# Autodesk Inventor assembly: Система подачи и забора проволоки
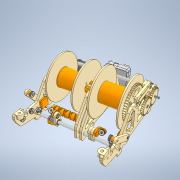
[picture p0: Inventor's stored thumbnail of the model, 180x180]
Saved by Autodesk Inventor 2021.1 (Build 251245010, 245A)
## iProperties
Created: 2026-04-13
Part Number: Система подачи и забора проволоки
Document SubType Name: Assembly
Designer: Андрей Тарасов
Author: Андрей Тарасов
## Documents named in this file (49)
- G:\04. Inventor\024. EDM 3.0\Система подачи и забора  проволоки\Система подачи и забора проволоки.iam
- G:\04. Inventor\024. EDM 3.0\Система подачи и забора  проволоки\Барабан катушки.ipt
- G:\04. Inventor\024. EDM 3.0\Система подачи и забора  проволоки\Бортик катушки.ipt
- G:\04. Inventor\024. EDM 3.0\Система подачи и забора  проволоки\Бортик внутренний.ipt
- G:\04. Inventor\024. EDM 3.0\Система подачи и забора  проволоки\Конусный барабан катушки.ipt
- G:\04. Inventor\024. EDM 3.0\Система подачи и забора  проволоки\Бортик конусной катушки.ipt
- G:\04. Inventor\024. EDM 3.0\Система подачи и забора  проволоки\Бортик внутренний (конусной катушки).ipt
- G:\04. Inventor\024. EDM 3.0\Система подачи и забора  проволоки\Вал катушки.ipt
- G:\04. Inventor\024. EDM 3.0\Система подачи и забора  проволоки\Опора катушки.ipt
- G:\04. Inventor\024. EDM 3.0\Система подачи и забора  проволоки\Опора катушки (врунтренняя).ipt
- G:\04. Inventor\024. EDM 3.0\Система подачи и забора  проволоки\Подшипник (8х12х3.5).ipt
- G:\04. Inventor\024. EDM 3.0\Система подачи и забора  проволоки\Вал шестерни.ipt
- G:\04. Inventor\024. EDM 3.0\Система подачи и забора  проволоки\Шестерня катушки.ipt
- G:\04. Inventor\024. EDM 3.0\Система подачи и забора  проволоки\Промежуточная шестерня (малая).ipt
- G:\04. Inventor\024. EDM 3.0\Система подачи и забора  проволоки\Рычаг фиксатора 1.ipt
- G:\04. Inventor\024. EDM 3.0\Система подачи и забора  проволоки\U-подшипник.ipt
- G:\04. Inventor\024. EDM 3.0\Система подачи и забора  проволоки\Рычаг натяжителя.ipt
- G:\04. Inventor\024. EDM 3.0\Система подачи и забора  проволоки\Петля ролика.ipt
- G:\04. Inventor\024. EDM 3.0\Система подачи и забора  проволоки\Крепление петли.ipt
- G:\04. Inventor\024. EDM 3.0\Система подачи и забора  проволоки\Крепление шкива.ipt
- G:\04. Inventor\024. EDM 3.0\Система подачи и забора  проволоки\Фиксатор трубки.ipt
- G:\04. Inventor\024. EDM 3.0\Система подачи и забора  проволоки\Трубка опоры (8 мм).ipt
- G:\04. Inventor\024. EDM 3.0\Система подачи и забора  проволоки\Петля ролика_MIR.ipt
- G:\04. Inventor\024. EDM 3.0\Система подачи и забора  проволоки\Линейный подшипник.ipt
- G:\04. Inventor\024. EDM 3.0\Система подачи и забора  проволоки\Крепление линейного подшипника.ipt
- G:\04. Inventor\024. EDM 3.0\Система подачи и забора  проволоки\Проставка катушки левая.ipt
- G:\04. Inventor\024. EDM 3.0\Система подачи и забора  проволоки\Проставка катушки правая.ipt
- G:\04. Inventor\024. EDM 3.0\Система подачи и забора  проволоки\Фиксатор левый.iam
- G:\04. Inventor\024. EDM 3.0\Система подачи и забора  проволоки\Фиксатор правый.iam
- G:\04. Inventor\024. EDM 3.0\Система подачи и забора  проволоки\Проставка шестерни.ipt
- G:\04. Inventor\024. EDM 3.0\Система подачи и забора  проволоки\Вал катушки (левой).ipt
- G:\04. Inventor\024. EDM 3.0\Система подачи и забора  проволоки\Вал шестерни (левой).ipt
- G:\04. Inventor\024. EDM 3.0\Система подачи и забора  проволоки\Проставка рычага натяжителя.ipt
- G:\04. Inventor\024. EDM 3.0\Система подачи и забора  проволоки\Бесконечный винт.ipt
- G:\04. Inventor\024. EDM 3.0\Система подачи и забора  проволоки\Бегунок.ipt
- G:\04. Inventor\024. EDM 3.0\Система подачи и забора  проволоки\Кольцо линейного подшипника.ipt
- G:\04. Inventor\024. EDM 3.0\Система подачи и забора  проволоки\Трубка винта.ipt
- G:\04. Inventor\024. EDM 3.0\Система подачи и забора  проволоки\AS5600.ipt
- G:\04. Inventor\024. EDM 3.0\Система подачи и забора  проволоки\Nema-17.ipt
- G:\04. Inventor\024. EDM 3.0\Система подачи и забора  проволоки\Шестерня мотора.ipt
- G:\04. Inventor\024. EDM 3.0\Система подачи и забора  проволоки\Шестерня промежуточная (большая).ipt
- G:\04. Inventor\024. EDM 3.0\Система подачи и забора  проволоки\Stepper 28BYJ-48.ipt
- G:\04. Inventor\024. EDM 3.0\Система подачи и забора  проволоки\Трубка рычага.ipt
- G:\04. Inventor\024. EDM 3.0\Система подачи и забора  проволоки\Шпунтик.ipt
- G:\04. Inventor\024. EDM 3.0\Система подачи и забора  проволоки\Шайба датчика.ipt
- G:\04. Inventor\024. EDM 3.0\Система подачи и забора  проволоки\Плата.ipt
- G:\04. Inventor\024. EDM 3.0\Система подачи и забора  проволоки\Корпус платы.ipt
- G:\04. Inventor\024. EDM 3.0\Система подачи и забора  проволоки\Крышка корпуса платы.ipt
- G:\04. Inventor\024. EDM 3.0\Колпачок датчика.ipt
## Components (93 placed, 48 different names)
1. Барабан катушки:1 — Совмещение:1, Совмещение:2, Заподлицо:1, Заподлицо:2, Совмещение:8, Совмещение:9
2. Бортик катушки:1 — Совмещение:1, Заподлицо:1, Заподлицо:6, Заподлицо:12, Совмещение:20, Совмещение:53, Совмещение:54
3. Бортик катушки:2 — Совмещение:2, Заподлицо:2, Заподлицо:7, Совмещение:63
4. Бортик катушки:3 — Совмещение:10, Заподлицо:8, Заподлицо:9, Совмещение:28, Совмещение:124, Заподлицо:50
5. Бортик внутренний:1 — Совмещение:12, Заподлицо:9, Совмещение:165
6. Бортик внутренний:2 — Совмещение:9, Заподлицо:7
7. Бортик внутренний:3 — Совмещение:8, Заподлицо:6, Совмещение:18
8. Конусный барабан катушки:1 — Совмещение:10, Заподлицо:8, Совмещение:12, Совмещение:15, Заподлицо:10, Совмещение:17
9. Бортик конусной катушки:1 — Совмещение:16, Совмещение:17, Совмещение:64
10. Бортик внутренний (конусной катушки):1 — Совмещение:15, Заподлицо:10, Совмещение:16
11. Вал катушки:1 — Совмещение:18, Заподлицо:12, Совмещение:22, Совмещение:52
12. Опора катушки:1 — Совмещение:20, Совмещение:22, Совмещение:46, Совмещение:47, Заподлицо:15, Заподлицо:16, Совмещение:73, Заподлицо:30, Совмещение:93, Совмещение:94, Совмещение:96, Совмещение:97, Совмещение:98, Совмещение:99, Совмещение:100, Заподлицо:31, Заподлицо:32, Совмещение:102, Совмещение:103, Совмещение:107, Заподлицо:33, Совмещение:111, Совмещение:145, Совмещение:164, Совмещение:206, Совмещение:207, Совмещение:212, Совмещение:216, Совмещение:217, Совмещение:220, Совмещение:221, Совмещение:238, Совмещение:244, Совмещение:247, Совмещение:248, Совмещение:259
13. Опора катушки:2 — Совмещение:28, Совмещение:44, Совмещение:45, Заподлицо:17, Заподлицо:18, Заподлицо:34, Заподлицо:37, Совмещение:119, Совмещение:120, Совмещение:140, Совмещение:141, Совмещение:142, Совмещение:146, Совмещение:154, Совмещение:155, Заподлицо:40, Совмещение:166, Совмещение:167, Совмещение:168, Совмещение:169, Совмещение:170, Совмещение:171, Совмещение:172, Совмещение:175, Заподлицо:42, Совмещение:176, Совмещение:177, Совмещение:190, Совмещение:195, Совмещение:196, Заподлицо:47, Заподлицо:49, Совмещение:204, Совмещение:209, Совмещение:210, Совмещение:213, Совмещение:218, Совмещение:219, Совмещение:222, Совмещение:223, Совмещение:229, Совмещение:231, Заподлицо:53, Совмещение:239, Совмещение:240, Совмещение:241, Заподлицо:58, Заподлицо:59, Совмещение:249, Совмещение:250, Совмещение:251, Совмещение:252, Совмещение:260
14. Подшипник (8х12х3.5):1 — Совмещение:46, Заподлицо:16
15. Подшипник (8х12х3.5):2 — Совмещение:47, Заподлицо:15, Совмещение:50
16. Подшипник (8х12х3.5):3 — Совмещение:44, Заподлицо:18
17. Подшипник (8х12х3.5):4 — Совмещение:45, Заподлицо:17, Совмещение:228
18. Вал шестерни:1 — Совмещение:50, Совмещение:51, Совмещение:54, Совмещение:227
19. Шестерня катушки:1 — Совмещение:52, Совмещение:53
20. Промежуточная шестерня (малая):1 — Совмещение:51, Совмещение:164
21. Опора катушки (врунтренняя):1 — Совмещение:64, Совмещение:109, Совмещение:139, Совмещение:143, Совмещение:144, Совмещение:150, Совмещение:197, Заподлицо:48, Совмещение:242, Совмещение:243, Совмещение:258, Заподлицо:60
22. Опора катушки (врунтренняя):2 — Совмещение:63, Совмещение:108, Совмещение:114, Совмещение:242
23. U-подшипник:1 — Совмещение:74, Совмещение:75
24. U-подшипник:2 — Совмещение:98, Совмещение:99
25. U-подшипник:3 — Совмещение:91, Совмещение:92
26. Подшипник (8х12х3.5):5 — Совмещение:100, Заподлицо:31, Совмещение:101
27. Рычаг натяжителя:1 — Совмещение:73, Совмещение:74, Совмещение:75, Совмещение:101, Совмещение:183, Совмещение:184, Совмещение:236, Заподлицо:56, Заподлицо:57
28. Петля ролика:1 — Совмещение:104, Совмещение:105, Совмещение:106, Совмещение:113
29. Крепление петли:1 — Совмещение:104, Совмещение:110, Совмещение:111, Совмещение:113, Совмещение:114, Совмещение:115, Заподлицо:35, Совмещение:117
30. U-подшипник:4 — Совмещение:105, Совмещение:106
31. Подшипник (8х12х3.5):6 — Совмещение:115, Заподлицо:35
32. Подшипник (8х12х3.5):7 — Совмещение:118, Заподлицо:36
33. Крепление шкива:1 — Совмещение:91, Совмещение:92, Заподлицо:30, Совмещение:93, Совмещение:94
34. U-подшипник:5 — Совмещение:96, Совмещение:97
35. Фиксатор трубки:1 — Заподлицо:32, Совмещение:102, Совмещение:103
36. Трубка опоры (8 мм):1 — Совмещение:107, Заподлицо:33, Совмещение:108, Совмещение:109, Заподлицо:34, Совмещение:110, Совмещение:116, Совмещение:131, Совмещение:204
37. Крепление петли:2 — Совмещение:116, Совмещение:117, Совмещение:118, Заподлицо:36
38. Крепление шкива:2 — Заподлицо:37, Совмещение:119, Совмещение:120, Совмещение:121, Совмещение:122
39. U-подшипник:6 — Совмещение:121, Совмещение:122
40. Шестерня катушки:2 — Совмещение:124, Совмещение:232
41. Петля ролика_MIR:1 — Совмещение:129, Совмещение:130, Совмещение:137, Совмещение:138
42. U-подшипник:7 — Совмещение:129, Совмещение:130
43. Линейный подшипник:1 — Совмещение:131, Совмещение:133, Совмещение:192, Заподлицо:44, Заподлицо:45
44. Крепление линейного подшипника:2 — Совмещение:133, Совмещение:137, Совмещение:138, Заподлицо:45, Совмещение:195, Совмещение:198, Заподлицо:46
45. Проставка катушки левая:1 — Совмещение:140, Совмещение:141, Совмещение:142
46. Проставка катушки правая:1 — Совмещение:139, Совмещение:143, Совмещение:144
47. Фиксатор левый:1 [sub-assembly] — Совмещение:145
48. Фиксатор правый:1 [sub-assembly] — Совмещение:146, Совмещение:156
49. Фиксатор левый:2 [sub-assembly] — Совмещение:150, Совмещение:151, Совмещение:152, Совмещение:153, Совмещение:253
50. Рычаг фиксатора 1:1 — Совмещение:151, Совмещение:152, Совмещение:153
51. Проставка шестерни:1 — Совмещение:154, Совмещение:155, Совмещение:156, Совмещение:160
52. Промежуточная шестерня (малая):2 — Совмещение:160
53. Вал катушки (левой):1 — Совмещение:165, Заподлицо:40, Совмещение:166, Совмещение:232
54. U-подшипник:8 — Совмещение:167, Совмещение:169
55. U-подшипник:9 — Совмещение:168, Совмещение:170
56. Рычаг натяжителя:2 — Совмещение:171, Совмещение:172, Совмещение:173, Совмещение:174, Совмещение:181, Совмещение:182, Совмещение:234, Заподлицо:54, Заподлицо:55
57. U-подшипник:10 — Совмещение:173, Совмещение:174
58. Подшипник (8х12х3.5):8 — Совмещение:175, Заподлицо:53
59. Фиксатор трубки:2 — Заподлицо:42, Совмещение:176, Совмещение:177
60. Вал шестерни (левой):1 — Совмещение:224, Совмещение:228, Заподлицо:52
61. Проставка рычага натяжителя:1 — Совмещение:181, Совмещение:182
62. Проставка рычага натяжителя:2 — Совмещение:183, Совмещение:184
63. Бесконечный винт:1 — Совмещение:190, Совмещение:193, Заподлицо:50
64. Бегунок:1 — Совмещение:193, Совмещение:194
65. Кольцо линейного подшипника:1 — Совмещение:192, Заподлицо:44, Совмещение:194
66. Подшипник (8х12х3.5):9 — Совмещение:196, Заподлицо:47, Совмещение:199
67. Подшипник (8х12х3.5):10 — Совмещение:198, Заподлицо:46
68. Подшипник (8х12х3.5):11 — Совмещение:197, Заподлицо:48
69. Трубка винта:1 — Совмещение:199, Заподлицо:49, Совмещение:230
70. AS5600:1 — Совмещение:206, Совмещение:207, Совмещение:238, Совмещение:245, Совмещение:246, Совмещение:263, Совмещение:264
71. AS5600:2 — Совмещение:209, Совмещение:210, Совмещение:239, Совмещение:261, Совмещение:262
72. Nema-17:1 — Совмещение:213, Совмещение:218, Совмещение:219, Совмещение:225
73. Nema-17:2 — Совмещение:212, Совмещение:216, Совмещение:217, Совмещение:226
74. Шестерня мотора:1 — Совмещение:221, Совмещение:226
75. Шестерня мотора:2 — Совмещение:222, Совмещение:225
76. Шестерня промежуточная (большая):1 — Совмещение:220, Совмещение:227
77. Шестерня промежуточная (большая):2 — Совмещение:223, Совмещение:224, Заподлицо:52
78. Stepper 28BYJ-48:1 — Совмещение:229, Совмещение:230, Совмещение:231
79. Трубка рычага:1 — Совмещение:236, Заподлицо:56, Совмещение:237
80. Шпунтик:1 — Заподлицо:55, Совмещение:235
81. Трубка рычага:2 — Совмещение:234, Заподлицо:54, Совмещение:235
82. Шпунтик:2 — Заподлицо:57, Совмещение:237
83. Трубка опоры (8 мм):2 — Совмещение:241, Заподлицо:59, Совмещение:243, Совмещение:244
84. Трубка опоры (8 мм):3 — Совмещение:240, Заподлицо:58, Совмещение:253
85. Шайба датчика:1 — Совмещение:250, Совмещение:252
86. Шайба датчика:2 — Совмещение:249, Совмещение:251
87. Шайба датчика:3 — Совмещение:245, Совмещение:247
88. Шайба датчика:4 — Совмещение:246, Совмещение:248
89. Плата:1 — Совмещение:254
90. Корпус платы:1 — Совмещение:254, Совмещение:255, Совмещение:256, Совмещение:257, Совмещение:258, Заподлицо:60
91. Крышка корпуса платы:1 — Совмещение:255, Совмещение:256, Совмещение:257
92. Колпачок датчика:1 — Совмещение:260, Совмещение:261, Совмещение:262
93. Колпачок датчика:2 — Совмещение:259, Совмещение:263, Совмещение:264
## Relationships (200: Mate 162, Flush 38)
- Совмещение:1 [Mate]: Барабан катушки:1 ↔ Бортик катушки:1
- Совмещение:2 [Mate]: Барабан катушки:1 ↔ Бортик катушки:2
- Заподлицо:1 [Flush]: Барабан катушки:1 ↔ Бортик катушки:1
- Заподлицо:2 [Flush]: Барабан катушки:1 ↔ Бортик катушки:2
- Совмещение:8 [Mate]: Барабан катушки:1 ↔ Бортик внутренний:3
- Совмещение:9 [Mate]: Барабан катушки:1 ↔ Бортик внутренний:2
- Заподлицо:6 [Flush]: Бортик катушки:1 ↔ Бортик внутренний:3
- Заподлицо:7 [Flush]: Бортик катушки:2 ↔ Бортик внутренний:2
- Совмещение:10 [Mate]: Бортик катушки:3 ↔ Конусный барабан катушки:1
- Заподлицо:8 [Flush]: Бортик катушки:3 ↔ Конусный барабан катушки:1
- Совмещение:12 [Mate]: Бортик внутренний:1 ↔ Конусный барабан катушки:1
- Заподлицо:9 [Flush]: Бортик катушки:3 ↔ Бортик внутренний:1
- Совмещение:15 [Mate]: Конусный барабан катушки:1 ↔ Бортик внутренний (конусной катушки):1
- Заподлицо:10 [Flush] (4 mm): Конусный барабан катушки:1 ↔ Бортик внутренний (конусной катушки):1
- Совмещение:16 [Mate]: Бортик конусной катушки:1 ↔ Бортик внутренний (конусной катушки):1
- Совмещение:17 [Mate]: Конусный барабан катушки:1 ↔ Бортик конусной катушки:1
- Совмещение:18 [Mate]: Бортик внутренний:3 ↔ Вал катушки:1
- Заподлицо:12 [Flush] (-13 mm): Бортик катушки:1 ↔ Вал катушки:1
- Совмещение:20 [Mate] (7 mm): Бортик катушки:1 ↔ Опора катушки:1
- Совмещение:22 [Mate]: Вал катушки:1 ↔ Опора катушки:1
- Совмещение:28 [Mate] (20 mm): Бортик катушки:3 ↔ Опора катушки:2
- Совмещение:44 [Mate]: Опора катушки:2 ↔ Подшипник (8х12х3.5):3
- Совмещение:45 [Mate]: Опора катушки:2 ↔ Подшипник (8х12х3.5):4
- Совмещение:46 [Mate]: Опора катушки:1 ↔ Подшипник (8х12х3.5):1
- Совмещение:47 [Mate]: Опора катушки:1 ↔ Подшипник (8х12х3.5):2
- Заподлицо:15 [Flush] (-0.5 mm): Опора катушки:1 ↔ Подшипник (8х12х3.5):2
- Заподлицо:16 [Flush] (-0.5 mm): Опора катушки:1 ↔ Подшипник (8х12х3.5):1
- Заподлицо:17 [Flush] (-0.5 mm): Опора катушки:2 ↔ Подшипник (8х12х3.5):4
- Заподлицо:18 [Flush] (-0.5 mm): Опора катушки:2 ↔ Подшипник (8х12х3.5):3
- Совмещение:50 [Mate]: Подшипник (8х12х3.5):2 ↔ Вал шестерни:1
- Совмещение:51 [Mate]: Вал шестерни:1 ↔ Промежуточная шестерня (малая):1
- Совмещение:52 [Mate]: Вал катушки:1 ↔ Шестерня катушки:1
- Совмещение:53 [Mate]: Бортик катушки:1 ↔ Шестерня катушки:1
- Совмещение:54 [Mate] (0.5 mm): Бортик катушки:1 ↔ Вал шестерни:1
- Совмещение:63 [Mate] (1 mm): Бортик катушки:2 ↔ Опора катушки (врунтренняя):2
- Совмещение:64 [Mate] (15 mm): Бортик конусной катушки:1 ↔ Опора катушки (врунтренняя):1
- Совмещение:73 [Mate] (0.5 mm): Опора катушки:1 ↔ Рычаг натяжителя:1
- Совмещение:74 [Mate]: U-подшипник:1 ↔ Рычаг натяжителя:1
- Совмещение:75 [Mate] (7 mm): U-подшипник:1 ↔ Рычаг натяжителя:1
- Совмещение:91 [Mate]: U-подшипник:3 ↔ Крепление шкива:1
- Совмещение:92 [Mate] (0.5 mm): U-подшипник:3 ↔ Крепление шкива:1
- Заподлицо:30 [Flush]: Опора катушки:1 ↔ Крепление шкива:1
- Совмещение:93 [Mate]: Опора катушки:1 ↔ Крепление шкива:1
- Совмещение:94 [Mate]: Опора катушки:1 ↔ Крепление шкива:1
- Совмещение:96 [Mate]: Опора катушки:1 ↔ U-подшипник:5
- Совмещение:97 [Mate] (0.5 mm): Опора катушки:1 ↔ U-подшипник:5
- Совмещение:98 [Mate]: Опора катушки:1 ↔ U-подшипник:2
- Совмещение:99 [Mate] (0.5 mm): Опора катушки:1 ↔ U-подшипник:2
- Совмещение:100 [Mate]: Опора катушки:1 ↔ Подшипник (8х12х3.5):5
- Заподлицо:31 [Flush]: Опора катушки:1 ↔ Подшипник (8х12х3.5):5
- Совмещение:101 [Mate]: Подшипник (8х12х3.5):5 ↔ Рычаг натяжителя:1
- Заподлицо:32 [Flush]: Опора катушки:1 ↔ Фиксатор трубки:1
- Совмещение:102 [Mate]: Опора катушки:1 ↔ Фиксатор трубки:1
- Совмещение:103 [Mate]: Опора катушки:1 ↔ Фиксатор трубки:1
- Совмещение:104 [Mate]: Петля ролика:1 ↔ Крепление петли:1
- Совмещение:105 [Mate]: Петля ролика:1 ↔ U-подшипник:4
- Совмещение:106 [Mate]: Петля ролика:1 ↔ U-подшипник:4
- Совмещение:107 [Mate]: Опора катушки:1 ↔ Трубка опоры (8 мм):1
- Заподлицо:33 [Flush]: Опора катушки:1 ↔ Трубка опоры (8 мм):1
- Совмещение:108 [Mate]: Опора катушки (врунтренняя):2 ↔ Трубка опоры (8 мм):1
- Совмещение:109 [Mate]: Опора катушки (врунтренняя):1 ↔ Трубка опоры (8 мм):1
- Заподлицо:34 [Flush]: Опора катушки:2 ↔ Трубка опоры (8 мм):1
- Совмещение:110 [Mate]: Крепление петли:1 ↔ Трубка опоры (8 мм):1
- Совмещение:111 [Mate]: Опора катушки:1 ↔ Крепление петли:1
- Совмещение:113 [Mate] (0.5 mm): Петля ролика:1 ↔ Крепление петли:1
- Совмещение:114 [Mate] (21 mm): Опора катушки (врунтренняя):2 ↔ Крепление петли:1
- Совмещение:115 [Mate]: Крепление петли:1 ↔ Подшипник (8х12х3.5):6
- Заподлицо:35 [Flush]: Крепление петли:1 ↔ Подшипник (8х12х3.5):6
- Совмещение:116 [Mate]: Трубка опоры (8 мм):1 ↔ Крепление петли:2
- Совмещение:117 [Mate]: Крепление петли:1 ↔ Крепление петли:2
- Совмещение:118 [Mate]: Подшипник (8х12х3.5):7 ↔ Крепление петли:2
- Заподлицо:36 [Flush]: Подшипник (8х12х3.5):7 ↔ Крепление петли:2
- Заподлицо:37 [Flush]: Опора катушки:2 ↔ Крепление шкива:2
- Совмещение:119 [Mate]: Опора катушки:2 ↔ Крепление шкива:2
- Совмещение:120 [Mate]: Опора катушки:2 ↔ Крепление шкива:2
- Совмещение:121 [Mate]: Крепление шкива:2 ↔ U-подшипник:6
- Совмещение:122 [Mate] (0.5 mm): Крепление шкива:2 ↔ U-подшипник:6
- Совмещение:124 [Mate]: Бортик катушки:3 ↔ Шестерня катушки:2
- Совмещение:129 [Mate]: Петля ролика_MIR:1 ↔ U-подшипник:7
- Совмещение:130 [Mate]: Петля ролика_MIR:1 ↔ U-подшипник:7
- Совмещение:131 [Mate]: Трубка опоры (8 мм):1 ↔ Линейный подшипник:1
- Совмещение:133 [Mate]: Линейный подшипник:1 ↔ Крепление линейного подшипника:2
- Совмещение:137 [Mate]: Петля ролика_MIR:1 ↔ Крепление линейного подшипника:2
- Совмещение:138 [Mate] (0.5 mm): Петля ролика_MIR:1 ↔ Крепление линейного подшипника:2
- Совмещение:139 [Mate]: Опора катушки (врунтренняя):1 ↔ Проставка катушки правая:1
- Совмещение:140 [Mate]: Опора катушки:2 ↔ Проставка катушки левая:1
- Совмещение:141 [Mate]: Опора катушки:2 ↔ Проставка катушки левая:1
- Совмещение:142 [Mate]: Опора катушки:2 ↔ Проставка катушки левая:1
- Совмещение:143 [Mate]: Опора катушки (врунтренняя):1 ↔ Проставка катушки правая:1
- Совмещение:144 [Mate]: Опора катушки (врунтренняя):1 ↔ Проставка катушки правая:1
- Совмещение:145 [Mate]: Опора катушки:1 ↔ Фиксатор левый:1
- Совмещение:146 [Mate]: Опора катушки:2 ↔ Фиксатор правый:1
- Совмещение:150 [Mate] (0.5 mm): Опора катушки (врунтренняя):1 ↔ Фиксатор левый:2
- Совмещение:151 [Mate]: Фиксатор левый:2 ↔ Рычаг фиксатора 1:1
- Совмещение:152 [Mate]: Фиксатор левый:2 ↔ Рычаг фиксатора 1:1
- Совмещение:153 [Mate]: Фиксатор левый:2 ↔ Рычаг фиксатора 1:1
- Совмещение:154 [Mate]: Опора катушки:2 ↔ Проставка шестерни:1
- Совмещение:155 [Mate]: Опора катушки:2 ↔ Проставка шестерни:1
- Совмещение:156 [Mate]: Фиксатор правый:1 ↔ Проставка шестерни:1
- Совмещение:160 [Mate] (0.5 mm): Проставка шестерни:1 ↔ Промежуточная шестерня (малая):2
- Совмещение:164 [Mate] (0.5 mm): Опора катушки:1 ↔ Промежуточная шестерня (малая):1
- Совмещение:165 [Mate]: Бортик внутренний:1 ↔ Вал катушки (левой):1
- Заподлицо:40 [Flush]: Опора катушки:2 ↔ Вал катушки (левой):1
- Совмещение:166 [Mate]: Опора катушки:2 ↔ Вал катушки (левой):1
- Совмещение:167 [Mate]: Опора катушки:2 ↔ U-подшипник:8
- Совмещение:168 [Mate]: Опора катушки:2 ↔ U-подшипник:9
- Совмещение:169 [Mate] (0.5 mm): Опора катушки:2 ↔ U-подшипник:8
- Совмещение:170 [Mate] (0.5 mm): Опора катушки:2 ↔ U-подшипник:9
- Совмещение:171 [Mate]: Опора катушки:2 ↔ Рычаг натяжителя:2
- Совмещение:172 [Mate] (0.5 mm): Опора катушки:2 ↔ Рычаг натяжителя:2
- Совмещение:173 [Mate] (7 mm): Рычаг натяжителя:2 ↔ U-подшипник:10
- Совмещение:174 [Mate]: Рычаг натяжителя:2 ↔ U-подшипник:10
- Совмещение:175 [Mate]: Опора катушки:2 ↔ Подшипник (8х12х3.5):8
- Заподлицо:42 [Flush]: Опора катушки:2 ↔ Фиксатор трубки:2
- Совмещение:176 [Mate]: Опора катушки:2 ↔ Фиксатор трубки:2
- Совмещение:177 [Mate]: Опора катушки:2 ↔ Фиксатор трубки:2
- Совмещение:181 [Mate]: Рычаг натяжителя:2 ↔ Проставка рычага натяжителя:1
- Совмещение:182 [Mate]: Рычаг натяжителя:2 ↔ Проставка рычага натяжителя:1
- Совмещение:183 [Mate]: Рычаг натяжителя:1 ↔ Проставка рычага натяжителя:2
- Совмещение:184 [Mate]: Рычаг натяжителя:1 ↔ Проставка рычага натяжителя:2
- Совмещение:190 [Mate]: Опора катушки:2 ↔ Бесконечный винт:1
- Совмещение:192 [Mate]: Линейный подшипник:1 ↔ Кольцо линейного подшипника:1
- Заподлицо:44 [Flush] (3 mm): Линейный подшипник:1 ↔ Кольцо линейного подшипника:1
- Совмещение:193 [Mate]: Бесконечный винт:1 ↔ Бегунок:1
- Совмещение:194 [Mate]: Бегунок:1 ↔ Кольцо линейного подшипника:1
- Заподлицо:45 [Flush]: Линейный подшипник:1 ↔ Крепление линейного подшипника:2
- Совмещение:195 [Mate]: Опора катушки:2 ↔ Крепление линейного подшипника:2
- Совмещение:196 [Mate]: Опора катушки:2 ↔ Подшипник (8х12х3.5):9
- Совмещение:197 [Mate]: Опора катушки (врунтренняя):1 ↔ Подшипник (8х12х3.5):11
- Совмещение:198 [Mate]: Крепление линейного подшипника:2 ↔ Подшипник (8х12х3.5):10
- Заподлицо:46 [Flush]: Крепление линейного подшипника:2 ↔ Подшипник (8х12х3.5):10
- Заподлицо:47 [Flush]: Опора катушки:2 ↔ Подшипник (8х12х3.5):9
- Заподлицо:48 [Flush]: Опора катушки (врунтренняя):1 ↔ Подшипник (8х12х3.5):11
- Совмещение:199 [Mate]: Подшипник (8х12х3.5):9 ↔ Трубка винта:1
- Заподлицо:49 [Flush]: Опора катушки:2 ↔ Трубка винта:1
- Заподлицо:50 [Flush] (-1 mm): Бортик катушки:3 ↔ Бесконечный винт:1
- Совмещение:204 [Mate]: Опора катушки:2 ↔ Трубка опоры (8 мм):1
- Совмещение:206 [Mate]: Опора катушки:1 ↔ AS5600:1
- Совмещение:207 [Mate]: Опора катушки:1 ↔ AS5600:1
- Совмещение:209 [Mate]: Опора катушки:2 ↔ AS5600:2
- Совмещение:210 [Mate]: Опора катушки:2 ↔ AS5600:2
- Совмещение:212 [Mate]: Опора катушки:1 ↔ Nema-17:2
- Совмещение:213 [Mate]: Опора катушки:2 ↔ Nema-17:1
- Совмещение:216 [Mate]: Опора катушки:1 ↔ Nema-17:2
- Совмещение:217 [Mate]: Опора катушки:1 ↔ Nema-17:2
- Совмещение:218 [Mate]: Опора катушки:2 ↔ Nema-17:1
- Совмещение:219 [Mate]: Опора катушки:2 ↔ Nema-17:1
- Совмещение:220 [Mate] (0.5 mm): Опора катушки:1 ↔ Шестерня промежуточная (большая):1
- Совмещение:221 [Mate] (0.5 mm): Опора катушки:1 ↔ Шестерня мотора:1
- Совмещение:222 [Mate] (0.5 mm): Опора катушки:2 ↔ Шестерня мотора:2
- Совмещение:223 [Mate] (0.5 mm): Опора катушки:2 ↔ Шестерня промежуточная (большая):2
- Совмещение:224 [Mate]: Вал шестерни (левой):1 ↔ Шестерня промежуточная (большая):2
- Совмещение:225 [Mate]: Nema-17:1 ↔ Шестерня мотора:2
- Совмещение:226 [Mate]: Nema-17:2 ↔ Шестерня мотора:1
- Совмещение:227 [Mate]: Вал шестерни:1 ↔ Шестерня промежуточная (большая):1
- Совмещение:228 [Mate]: Подшипник (8х12х3.5):4 ↔ Вал шестерни (левой):1
- Заподлицо:52 [Flush]: Вал шестерни (левой):1 ↔ Шестерня промежуточная (большая):2
- Совмещение:229 [Mate]: Опора катушки:2 ↔ Stepper 28BYJ-48:1
- Совмещение:230 [Mate]: Трубка винта:1 ↔ Stepper 28BYJ-48:1
- Совмещение:231 [Mate]: Опора катушки:2 ↔ Stepper 28BYJ-48:1
- Совмещение:232 [Mate]: Шестерня катушки:2 ↔ Вал катушки (левой):1
- Заподлицо:53 [Flush]: Опора катушки:2 ↔ Подшипник (8х12х3.5):8
- Совмещение:234 [Mate]: Рычаг натяжителя:2 ↔ Трубка рычага:2
- Заподлицо:54 [Flush]: Рычаг натяжителя:2 ↔ Трубка рычага:2
- Заподлицо:55 [Flush]: Рычаг натяжителя:2 ↔ Шпунтик:1
- Совмещение:235 [Mate]: Шпунтик:1 ↔ Трубка рычага:2
- Совмещение:236 [Mate]: Рычаг натяжителя:1 ↔ Трубка рычага:1
- Заподлицо:56 [Flush]: Рычаг натяжителя:1 ↔ Трубка рычага:1
- Заподлицо:57 [Flush]: Рычаг натяжителя:1 ↔ Шпунтик:2
- Совмещение:237 [Mate]: Трубка рычага:1 ↔ Шпунтик:2
- Совмещение:238 [Mate] (1 mm): Опора катушки:1 ↔ AS5600:1
- Совмещение:239 [Mate] (1 mm): Опора катушки:2 ↔ AS5600:2
- Совмещение:240 [Mate]: Опора катушки:2 ↔ Трубка опоры (8 мм):3
- Совмещение:241 [Mate]: Опора катушки:2 ↔ Трубка опоры (8 мм):2
- Заподлицо:58 [Flush]: Опора катушки:2 ↔ Трубка опоры (8 мм):3
- Заподлицо:59 [Flush]: Опора катушки:2 ↔ Трубка опоры (8 мм):2
- Совмещение:242 [Mate]: Опора катушки (врунтренняя):1 ↔ Опора катушки (врунтренняя):2
- Совмещение:243 [Mate]: Опора катушки (врунтренняя):1 ↔ Трубка опоры (8 мм):2
- Совмещение:244 [Mate]: Опора катушки:1 ↔ Трубка опоры (8 мм):2
- Совмещение:245 [Mate]: AS5600:1 ↔ Шайба датчика:3
- Совмещение:246 [Mate]: AS5600:1 ↔ Шайба датчика:4
- Совмещение:247 [Mate]: Опора катушки:1 ↔ Шайба датчика:3
- Совмещение:248 [Mate]: Опора катушки:1 ↔ Шайба датчика:4
- Совмещение:249 [Mate]: Опора катушки:2 ↔ Шайба датчика:2
- Совмещение:250 [Mate]: Опора катушки:2 ↔ Шайба датчика:1
- Совмещение:251 [Mate]: Опора катушки:2 ↔ Шайба датчика:2
- Совмещение:252 [Mate]: Опора катушки:2 ↔ Шайба датчика:1
- Совмещение:253 [Mate]: Фиксатор левый:2 ↔ Трубка опоры (8 мм):3
- Совмещение:254 [Mate]: Плата:1 ↔ Корпус платы:1
- Совмещение:255 [Mate] (0.1 mm): Корпус платы:1 ↔ Крышка корпуса платы:1
- Совмещение:256 [Mate] (0.1 mm): Корпус платы:1 ↔ Крышка корпуса платы:1
- Совмещение:257 [Mate]: Корпус платы:1 ↔ Крышка корпуса платы:1
- Совмещение:258 [Mate]: Опора катушки (врунтренняя):1 ↔ Корпус платы:1
- Заподлицо:60 [Flush] (5 mm): Опора катушки (врунтренняя):1 ↔ Корпус платы:1
- Совмещение:259 [Mate]: Опора катушки:1 ↔ Колпачок датчика:2
- Совмещение:260 [Mate]: Опора катушки:2 ↔ Колпачок датчика:1
- Совмещение:261 [Mate]: AS5600:2 ↔ Колпачок датчика:1
- Совмещение:262 [Mate]: AS5600:2 ↔ Колпачок датчика:1
- Совмещение:263 [Mate]: AS5600:1 ↔ Колпачок датчика:2
- Совмещение:264 [Mate]: AS5600:1 ↔ Колпачок датчика:2
